# Autodesk Inventor assembly: TS_Positionierungseinheit_Rahmen_int
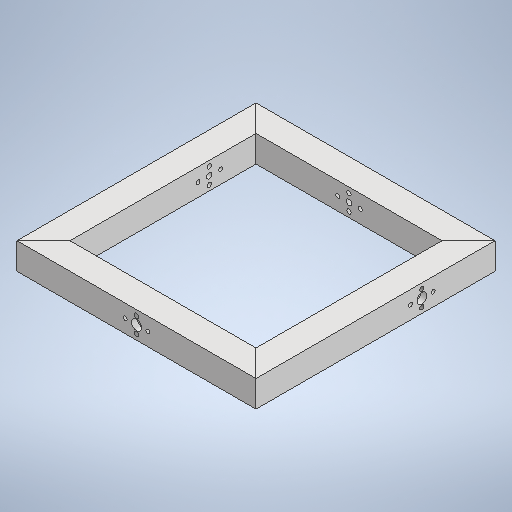
[picture p0: Inventor's stored thumbnail of the model, 512x512]
Saved by Autodesk Inventor 2025.1 (Build 291241000, 241)
## iProperties
Created: 2025-05-23
Part Number: TS_Positionierungseinheit_Rahmen_int
Document SubType Name: Weldment
Designer: tino
Weld Material: Welded Aluminum-6061
Author: tino
## Documents named in this file (3)
- C:\Users\Erik\Erik\Hochschule\3. Semester\CAD\Useless Box\Eigene Bauteile\TS_Positionierungseinheit_Rahmen_int.iam
- C:\Users\Erik\Erik\Hochschule\3. Semester\CAD\Useless Box\Eigene Bauteile\TS_Positionierungseinheit_Rahmen_int.ipt
- C:\Users\Erik\Erik\Hochschule\3. Semester\CAD\Useless Box\Eigene Bauteile\TS_Positionierungseinheit_Rahmen_exzentrisch_int.ipt
## Components (4 placed, 2 different names)
1. TS_Positionierungseinheit_Rahmen_int:5 — Mate:3, Flush:2, Mate:4, Mate:6, Symmetry:2, Symmetry:3
2. TS_Positionierungseinheit_Rahmen_int:7 — Mate:1, Flush:1, Mate:2, Mate:5, Flush:3, Symmetry:2
3. TS_Positionierungseinheit_Rahmen_exzentrisch_int:1 — Mate:5, Mate:6, Flush:3, Symmetry:1
4. TS_Positionierungseinheit_Rahmen_exzentrisch_int:2 — Mate:1, Flush:1, Mate:2, Mate:3, Flush:2, Mate:4, Symmetry:1, Symmetry:3
## Relationships (14: Mate 8, Flush 3, Symmetry 3)
- Mate:1: TS_Positionierungseinheit_Rahmen_int:7 ↔ TS_Positionierungseinheit_Rahmen_exzentrisch_int:2
- Flush:1: TS_Positionierungseinheit_Rahmen_int:7 ↔ TS_Positionierungseinheit_Rahmen_exzentrisch_int:2
- Mate:2: TS_Positionierungseinheit_Rahmen_int:7 ↔ TS_Positionierungseinheit_Rahmen_exzentrisch_int:2
- Mate:3: TS_Positionierungseinheit_Rahmen_int:5 ↔ TS_Positionierungseinheit_Rahmen_exzentrisch_int:2
- Flush:2: TS_Positionierungseinheit_Rahmen_int:5 ↔ TS_Positionierungseinheit_Rahmen_exzentrisch_int:2
- Mate:4: TS_Positionierungseinheit_Rahmen_int:5 ↔ TS_Positionierungseinheit_Rahmen_exzentrisch_int:2
- Mate:5: TS_Positionierungseinheit_Rahmen_int:7 ↔ TS_Positionierungseinheit_Rahmen_exzentrisch_int:1
- Mate:6: TS_Positionierungseinheit_Rahmen_int:5 ↔ TS_Positionierungseinheit_Rahmen_exzentrisch_int:1
- Flush:3: TS_Positionierungseinheit_Rahmen_int:7 ↔ TS_Positionierungseinheit_Rahmen_exzentrisch_int:1
- Symmetry:1: TS_Positionierungseinheit_Rahmen_exzentrisch_int:1 ↔ TS_Positionierungseinheit_Rahmen_exzentrisch_int:2
- Symmetry:2: TS_Positionierungseinheit_Rahmen_int:5 ↔ TS_Positionierungseinheit_Rahmen_int:7
- Mate:7
- Mate:8
- Symmetry:3: TS_Positionierungseinheit_Rahmen_int:5 ↔ TS_Positionierungseinheit_Rahmen_exzentrisch_int:2
